# Autodesk Inventor assembly: motor with bevel pinion gear
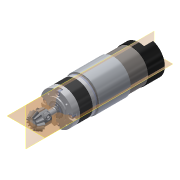
[picture p0: Inventor's stored thumbnail of the model, 180x180]
Saved by Autodesk Inventor 2018 (Build 220112000, 112)
## iProperties
Created: 2019-09-29
Part Number: motor with bevel pinion gear
Document SubType Name: Assembly
Designer: ball
Author: ball
## Documents named in this file (3)
- C:\FTC\FTC8863CAD\2019 Robot\Mecanum Drive Train\motor with bevel pinion gear.iam
- C:\FTC\FTC8863CAD\Andymark\am-3461a+NeveRest+Orbital+3.7+REV2.ipt
- C:\FTC\FTC8863CAD\Actobotics\615 parts\615458 assembly.ipt
## Components (2 placed, 2 different names)
1. am-3461a+NeveRest+Orbital+3.7+REV2:1 — Mate:1, Flush:1, Mate:2, Mate:3
2. 615458 assembly:1 — Mate:1, Flush:1
## Relationships (4: Mate 3, Flush 1)
- Mate:1: am-3461a+NeveRest+Orbital+3.7+REV2:1 ↔ 615458 assembly:1
- Flush:1: am-3461a+NeveRest+Orbital+3.7+REV2:1 ↔ 615458 assembly:1
- Mate:2: am-3461a+NeveRest+Orbital+3.7+REV2:1
- Mate:3: am-3461a+NeveRest+Orbital+3.7+REV2:1
